# Autodesk Inventor assembly: Ensamblaje1
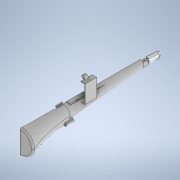
[picture p0: Inventor's stored thumbnail of the model, 180x180]
Saved by Autodesk Inventor 2021 (Build 250183000, 183)
## iProperties
Created: 2023-07-31
Part Number: Ensamblaje1
Document SubType Name: Assembly
Designer: Sergio
Author: Sergio
## Documents named in this file (17)
- D:\Sergio\OneDrive - Escuela Superior Politécnica del Litoral\Documentos\12vo Semestre (último)\Diseño Mecatrónico\Proyecto\Diseño Mecánico\solucion GANADORA\Ensamblaje1.iam
- D:\Sergio\OneDrive - Escuela Superior Politécnica del Litoral\Documentos\12vo Semestre (último)\Diseño Mecatrónico\Proyecto\Diseño Mecánico\solucion GANADORA\Base.ipt
- D:\Sergio\OneDrive - Escuela Superior Politécnica del Litoral\Documentos\12vo Semestre (último)\Diseño Mecatrónico\Proyecto\Diseño Mecánico\solucion GANADORA\dedo\finger_solid_joint.ipt
- D:\Sergio\OneDrive - Escuela Superior Politécnica del Litoral\Documentos\12vo Semestre (último)\Diseño Mecatrónico\Proyecto\Diseño Mecánico\solucion GANADORA\dedo\celda de carga.ipt
- D:\Sergio\OneDrive - Escuela Superior Politécnica del Litoral\Documentos\12vo Semestre (último)\Diseño Mecatrónico\Proyecto\Diseño Mecánico\solucion GANADORA\trigger_mechanism\link_connector.ipt
- D:\Sergio\OneDrive - Escuela Superior Politécnica del Litoral\Documentos\12vo Semestre (último)\Diseño Mecatrónico\Proyecto\Diseño Mecánico\solucion GANADORA\trigger_mechanism\link3.ipt
- D:\Sergio\OneDrive - Escuela Superior Politécnica del Litoral\Documentos\12vo Semestre (último)\Diseño Mecatrónico\Proyecto\Diseño Mecánico\solucion GANADORA\trigger_mechanism\trigger.ipt
- D:\Sergio\Documents\Inventor\Content Center Files\R2021\es-ES\AS 1427(00)\AS 1427 - M4 x 16(4).ipt
- D:\Sergio\OneDrive - Escuela Superior Politécnica del Litoral\Documentos\12vo Semestre (último)\Diseño Mecatrónico\Proyecto\Diseño Mecánico\solucion GANADORA\dedo\flexible.ipt
- D:\Sergio\OneDrive - Escuela Superior Politécnica del Litoral\Documentos\12vo Semestre (último)\Diseño Mecatrónico\Proyecto\Diseño Mecánico\solucion GANADORA\link_4.ipt
- D:\Sergio\OneDrive - Escuela Superior Politécnica del Litoral\Documentos\12vo Semestre (último)\Diseño Mecatrónico\Proyecto\Diseño Mecánico\solucion GANADORA\dedo\finger_solid_upsection.ipt
- D:\Sergio\OneDrive - Escuela Superior Politécnica del Litoral\Documentos\12vo Semestre (último)\Diseño Mecatrónico\Proyecto\Diseño Mecánico\solucion GANADORA\dedo\shaft_finger_r4.ipt
- D:\Sergio\Documents\Inventor\Content Center Files\R2021\es-ES\AS 1427(04)\AS 1427 - M2 x 8(5) I.ipt
- D:\Sergio\OneDrive - Escuela Superior Politécnica del Litoral\Documentos\12vo Semestre (último)\Diseño Mecatrónico\Proyecto\Diseño Mecánico\solucion GANADORA\trigger_mechanism\link\shaft_bar.ipt
- D:\Sergio\Documents\Inventor\Content Center Files\R2021\es-ES\BS 4183(2)\BS 4183 - M4 x 16(1) I.ipt
- D:\Sergio\OneDrive - Escuela Superior Politécnica del Litoral\Documentos\12vo Semestre (último)\Diseño Mecatrónico\Proyecto\Diseño Mecánico\solucion GANADORA\Caja.ipt
- D:\Sergio\OneDrive - Escuela Superior Politécnica del Litoral\Documentos\12vo Semestre (último)\Diseño Mecatrónico\Proyecto\Diseño Mecánico\solucion GANADORA\parameters.xlsx
## Components (15 placed, 15 different names)
1. Base:1 — Coincidencia:1, Coincidencia:3, Coincidencia:4, Coincidencia:5, Coincidencia:34, Coincidencia:7, Coincidencia:25, Coincidencia:26, Coincidencia:33, Nivelación:2, Nivelación:39
2. finger_solid_joint:1 — Coincidencia:12, Coincidencia:14, Coincidencia:25, Coincidencia:26, Coincidencia:27, Nivelación:3
3. celda de carga:1 — Coincidencia:17, Coincidencia:18, Coincidencia:19
4. link_connector:1 — Coincidencia:4, Coincidencia:5, Insertar:2, Coincidencia:35
5. link3:1 — Coincidencia:35, Coincidencia:36, Coincidencia:37
6. trigger:1 — Coincidencia:3, Coincidencia:34, Coincidencia:36, Coincidencia:37
7. AS 1427 - Métrico M4 x 16:1 — Coincidencia:1, Coincidencia:7
8. finger_solid_upsection:1 — Coincidencia:16, Coincidencia:18, Coincidencia:19, Insertar:1, Coincidencia:27, Coincidencia:28, Nivelación:1
9. shaft_finger_r4:1 — Coincidencia:12, Tangente:4, Nivelación:3
10. BS 4183 Tornillo para maquinaria de cabeza plana avellanada con hueco cruciforme - Métrico M4 x 16:1 — Coincidencia:14, Insertar:1
11. AS 1427 H - Métrico M2 x 8:1 — Coincidencia:16, Coincidencia:17
12. flexible:1 — Coincidencia:28, Nivelación:1
13. link_4:1 — Tangente:4, Tangente:5, Coincidencia:33
14. shaft_bar:1 — Insertar:2, Tangente:5
15. Caja:1 — Nivelación:39
## Relationships (28: Mate 20, Flush 4, Insert 2, Tangent 2)
- Coincidencia:1 [Mate]: Base:1 ↔ AS 1427 - Métrico M4 x 16:1
- Coincidencia:3 [Mate]: Base:1 ↔ trigger:1
- Coincidencia:4 [Mate]: Base:1 ↔ link_connector:1
- Coincidencia:5 [Mate] (0.5 mm): Base:1 ↔ link_connector:1
- Coincidencia:34 [Mate]: Base:1 ↔ trigger:1
- Coincidencia:7 [Mate]: Base:1 ↔ AS 1427 - Métrico M4 x 16:1
- Coincidencia:12 [Mate]: finger_solid_joint:1 ↔ shaft_finger_r4:1
- Coincidencia:14 [Mate]: finger_solid_joint:1 ↔ BS 4183 Tornillo para maquinaria de cabeza plana avellanada con hueco cruciforme - Métrico M4 x 16:1
- Coincidencia:16 [Mate]: finger_solid_upsection:1 ↔ AS 1427 H - Métrico M2 x 8:1
- Coincidencia:17 [Mate]: celda de carga:1 ↔ AS 1427 H - Métrico M2 x 8:1
- Coincidencia:18 [Mate]: celda de carga:1 ↔ finger_solid_upsection:1
- Coincidencia:19 [Mate]: celda de carga:1 ↔ finger_solid_upsection:1
- Insertar:1: finger_solid_upsection:1 ↔ BS 4183 Tornillo para maquinaria de cabeza plana avellanada con hueco cruciforme - Métrico M4 x 16:1
- Coincidencia:25 [Mate]: Base:1 ↔ finger_solid_joint:1
- Coincidencia:26 [Mate]: Base:1 ↔ finger_solid_joint:1
- Coincidencia:27 [Mate]: finger_solid_joint:1 ↔ finger_solid_upsection:1
- Coincidencia:28 [Mate]: finger_solid_upsection:1 ↔ flexible:1
- Insertar:2: link_connector:1 ↔ shaft_bar:1
- Tangente:4: shaft_finger_r4:1 ↔ link_4:1
- Tangente:5: link_4:1 ↔ shaft_bar:1
- Coincidencia:33 [Mate]: Base:1 ↔ link_4:1
- Nivelación:1 [Flush]: finger_solid_upsection:1 ↔ flexible:1
- Nivelación:2 [Flush] (-80 mm): Base:1
- Nivelación:3 [Flush]: finger_solid_joint:1 ↔ shaft_finger_r4:1
- Coincidencia:35 [Mate]: link_connector:1 ↔ link3:1
- Coincidencia:36 [Mate]: link3:1 ↔ trigger:1
- Coincidencia:37 [Mate]: link3:1 ↔ trigger:1
- Nivelación:39 [Flush]: Base:1 ↔ Caja:1
## Named parameters: offset = 1 mm, thikness = 2 mm, r1 = 5.55 mm, r2o = 59.75 mm, delta_y = 6 mm, r4 = 60 mm, wire_d = 1 mm, vueltas = 4, width_ang_spring = 5 mm, spring_int_diam = 8.5 mm, spring_ext_diam = 10.5 mm, r3 = 8.25 mm, r3R = 4.75 mm, r3T = 6.74537 mm, alpha = 54.847297 deg, alpha2 = 270 deg, theta3_recogido = 305.152703 deg, delta_theta_3 = 45 deg, joint_width = 12 mm, joint_radius = 7.75 mm, shaft_width = 15 mm, shaft_joint_diameter = 7.75 mm, separation_space = 0.5 mm, height_finger = 42 mm, width_finger = 20 mm, cell_screw_head_diameter = 4 mm, cell_screw_diameter = 2 mm, cell_space = 2 mm, cell_width = 6 mm, cell_theta_position = 60 deg, cell_thikness = 1 mm, cell_lenght = 37 mm, cell_z_space = 5 mm, secure_distance = 250 mm, hand_lenght = 110 mm, hand_space = 30 mm, wire_D = 2.3 mm, width_link = 8 mm, Dt = 1.05949 mm, Djoint_shaft = 2.3 mm, shaft_x = 1.45 mm, shaft_y = 6.45 mm, lenght_body_link = 186.05 mm, lenght_bar_support = 201.65 mm, wire_spring_d = 1 mm, spring_int_d = 6 mm, spring_lenght = 28 mm, trigger_offset = 2 mm, m2_theta2o = 107 deg, m2_r2 = 28 mm, e = 9 mm, So = 17 mm, m2_theta3o = -30 deg, m2_r3 = 19.75 mm, m2_delta_theta1 = 15 deg, m2_theta3f = -60 deg, trigger_thumb_lenght = 6 mm, width_r12 = 8 mm, width_r3 = 10 mm, m2_r1 = 25.2 mm, m2_r1_down_width = 20 mm, r3_thikness = 3.5 mm, t_thikness = 3 mm, t_thikness2 = 10 mm, tg_lenght = 30 mm, tg_width = 4 mm, pivot_screw_d = 4 mm, pivot_diameter = 7 mm, sj_diam_shaft = 6 mm, sj_groove = 2 mm, sj_groove_deep = 7 mm, sj_head_D = 7 mm, sj_head_d = 4.7464 mm, sj_head_height = 5 mm, sf_lenght = 9.5 mm, sf_base = 3 mm, sf_head_height = 3 mm, sf_head_width = 4.5 mm, sf_head_offset = 0.25 mm, sf_head_grip_width = 2 mm, sf_head_angle = 45 deg, sf_thikness = 5 mm, screw_Dhead = 8 mm, screw_d = 4 mm, screw_lenght = 12 mm, screwJ_base_D = 9 mm, screwJ_top_D = 13 mm, gj_D = 6 mm, gj_d = 4 mm, gj_out_section = 6 mm, ext_width_slider = 3.5 mm, sfbox_tip_width = 2.5 mm, slim_width_slider = 1.5 mm, agarradera_width = 4 mm, int_width_slider = 2 mm, agarradera_position = 40.13077 mm, sfbox_theta1 = 60 deg, sfbox_theta2 = 45 deg, agarradera_theta = 60 deg, sfbox_width = 1.5 mm, box_fat_slider_lenght = 35 mm, fat_width_slider = 2 mm, box_in_width = 55 mm, flex_separation_theta = 60 deg, offset_base_box = 19 mm, sf_flex_separation = 17.66667 mm, thikness_box = 1.5 mm, box_slim_slider_lenght = 53 mm, box_base_lenght = 57 mm, box_in_deep = 35 mm, box_separation = 10 mm, box_in_height = 55 mm, box_base_width = 24 mm
